# Autodesk Inventor assembly: bras_main
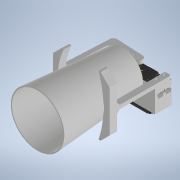
[picture p0: Inventor's stored thumbnail of the model, 180x180]
Saved by Autodesk Inventor 2020 (Build 240168000, 168)
## iProperties
Created: 2019-12-27
Part Number: bras_main
Document SubType Name: Assembly
Designer: bapti
Author: bapti
## Documents named in this file (6)
- C:\Users\bapti\Documents\EIRBOT\eirbot2020-2A\Meca\EIRBOT_sailtheworld\robot\bras\bras_main.iam
- C:\Users\bapti\Documents\EIRBOT\eirbot2020-2A\Meca\EIRBOT_sailtheworld\mg995\MG_996R.iam
- C:\Users\bapti\Documents\EIRBOT\eirbot2020-2A\Meca\EIRBOT_sailtheworld\board\boue.ipt
- C:\Users\bapti\Documents\EIRBOT\eirbot2020-2A\Meca\EIRBOT_sailtheworld\robot\bras\pince_mouvante.ipt
- C:\Users\bapti\Documents\EIRBOT\eirbot2020-2A\Meca\EIRBOT_sailtheworld\robot\bras\pince_statique.ipt
- C:\Users\bapti\Documents\EIRBOT\eirbot2020-2A\Meca\EIRBOT_sailtheworld\robot\bras\pince_statique_1.ipt
## Components (5 placed, 5 different names)
1. MG_996R:1 [sub-assembly] — Affleurement:1, Affleurement:2, Affleurement:3, Placage:4, Placage:5, Placage:7, Placage:8, Placage:9
2. boue:1
3. pince_mouvante:1 — Placage:4, Placage:5
4. pince_statique:1 — Placage:6, Placage:7, Placage:8, Placage:9, Placage:10, Placage:11
5. pince_statique_1:1 — Placage:6, Placage:10, Placage:11
## Relationships (11: Mate 8, Flush 3)
- Affleurement:1 [Flush]: MG_996R:1
- Affleurement:2 [Flush]: MG_996R:1
- Affleurement:3 [Flush]: MG_996R:1
- Placage:4 [Mate]: MG_996R:1 ↔ pince_mouvante:1
- Placage:5 [Mate]: MG_996R:1 ↔ pince_mouvante:1
- Placage:6 [Mate]: pince_statique:1 ↔ pince_statique_1:1
- Placage:7 [Mate]: MG_996R:1 ↔ pince_statique:1
- Placage:8 [Mate]: MG_996R:1 ↔ pince_statique:1
- Placage:9 [Mate]: MG_996R:1 ↔ pince_statique:1
- Placage:10 [Mate]: pince_statique:1 ↔ pince_statique_1:1
- Placage:11 [Mate]: pince_statique:1 ↔ pince_statique_1:1
